# Autodesk Inventor assembly: Katze
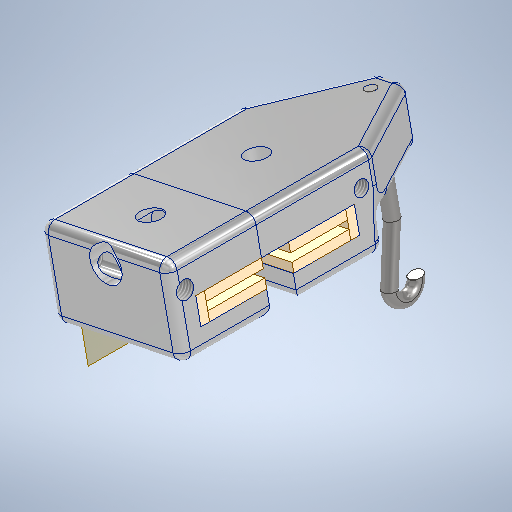
[picture p0: Inventor's stored thumbnail of the model, 512x512]
Saved by Autodesk Inventor 2025 (Build 290162010, 162A)
## iProperties
Created: 2024-11-19
Part Number: Katze
Document SubType Name: Assembly
Designer: Admin
Mass: 66.181 g
Surface Area: 161.129 cm^2
Volume: 25.2769 cm^3
Density: 2.61824 g/cm^3
Author: Admin
## Documents named in this file (6)
- C:\Users\Admin\GIT\HDVKBM\CAD\Krandemonstrator\KatzeFEM.iam
- C:\Users\Admin\GIT\HDVKBM\CAD\Krandemonstrator\Katze_Lagerhalter_hinten.ipt
- C:\Users\Admin\GIT\HDVKBM\CAD\Krandemonstrator\Katze_Lagerhalter_vorne.ipt
- C:\Users\Admin\GIT\HDVKBM\CAD\Krandemonstrator\LagerHH.ipt
- C:\Users\Admin\GIT\HDVKBM\CAD\Krandemonstrator\LagerHO.ipt
- C:\Users\Admin\GIT\HDVKBM\CAD\Krandemonstrator\M3 Haken 40mm.ipt
## Components (9 placed, 5 different names)
1. Katze_Lagerhalter_hinten:1 — Planar:1, Planar:2, Planar:3, Planar:5
2. Katze_Lagerhalter_vorne:1 — Planar:7, Planar:8, Planar:10, Planar:12, Starr:13
3. LagerHH:1 — Planar:1, Planar:2, Planar:4, Planar:6
4. LagerHH:2 — Planar:7, Planar:8, Planar:11, Planar:13
5. LagerHO:1 — Planar:10, Planar:11
6. LagerHO:2 — Planar:5, Planar:6
7. LagerHO:3 — Planar:3, Planar:4
8. LagerHO:4 — Planar:12, Planar:13
9. M3 Haken 40mm:1 — Starr:13
## Relationships (13: PlanarJoint 12, WeldJoint 1)
- Planar:1: Katze_Lagerhalter_hinten:1 ↔ LagerHH:1
- Planar:2: Katze_Lagerhalter_hinten:1 ↔ LagerHH:1
- Planar:3: Katze_Lagerhalter_hinten:1 ↔ LagerHO:3
- Planar:4: LagerHH:1 ↔ LagerHO:3
- Planar:5: Katze_Lagerhalter_hinten:1 ↔ LagerHO:2
- Planar:6: LagerHH:1 ↔ LagerHO:2
- Planar:7: Katze_Lagerhalter_vorne:1 ↔ LagerHH:2
- Planar:8: Katze_Lagerhalter_vorne:1 ↔ LagerHH:2
- Planar:10: Katze_Lagerhalter_vorne:1 ↔ LagerHO:1
- Planar:11: LagerHH:2 ↔ LagerHO:1
- Planar:12: Katze_Lagerhalter_vorne:1 ↔ LagerHO:4
- Planar:13: LagerHH:2 ↔ LagerHO:4
- Starr:13 [WeldJoint]: Katze_Lagerhalter_vorne:1 ↔ M3 Haken 40mm:1
